# Autodesk Inventor assembly: 900-10-WHEEL-ASM-01
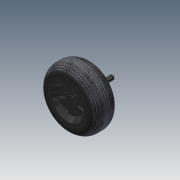
[picture p0: Inventor's stored thumbnail of the model, 180x180]
Saved by Autodesk Inventor 2018.2 (Build 222227000, 227)
## iProperties
Created: 2017-10-25
Part Number: 900-10-WHEEL-ASM-01
Document SubType Name: Assembly
Designer: marti
Author: marti
## Documents named in this file (4)
- D:\Programmierung\FRANC0R\CAD\02-Rocker-Bogie-Robot\900-COMPONENTS\900-10-WHEEL\900-10-WHEEL-ASM-01.iam
- D:\Programmierung\FRANC0R\CAD\02-Rocker-Bogie-Robot\900-COMPONENTS\900-10-WHEEL\900-10-WHEEL-03.ipt
- D:\Programmierung\FRANC0R\CAD\02-Rocker-Bogie-Robot\900-COMPONENTS\900-10-WHEEL\900-10-WHEEL-01.ipt
- D:\Programmierung\FRANC0R\CAD\02-Rocker-Bogie-Robot\900-COMPONENTS\900-10-WHEEL\900-10-WHEEL-02.ipt
## Components (3 placed, 3 different names)
1. 900-10-WHEEL-03:1 — Passend:1, Passend:2
2. 900-10-WHEEL-01:1 — Passend:1, Passend:2, Passend:3, Passend:5, Passend:6
3. 900-10-WHEEL-02:1 — Passend:3, Passend:5, Passend:6
## Relationships (5: Mate 5)
- Passend:1 [Mate]: 900-10-WHEEL-03:1 ↔ 900-10-WHEEL-01:1
- Passend:2 [Mate]: 900-10-WHEEL-03:1 ↔ 900-10-WHEEL-01:1
- Passend:3 [Mate]: 900-10-WHEEL-01:1 ↔ 900-10-WHEEL-02:1
- Passend:5 [Mate]: 900-10-WHEEL-01:1 ↔ 900-10-WHEEL-02:1
- Passend:6 [Mate]: 900-10-WHEEL-01:1 ↔ 900-10-WHEEL-02:1
